# Autodesk Inventor assembly: Assembly_miscelatore
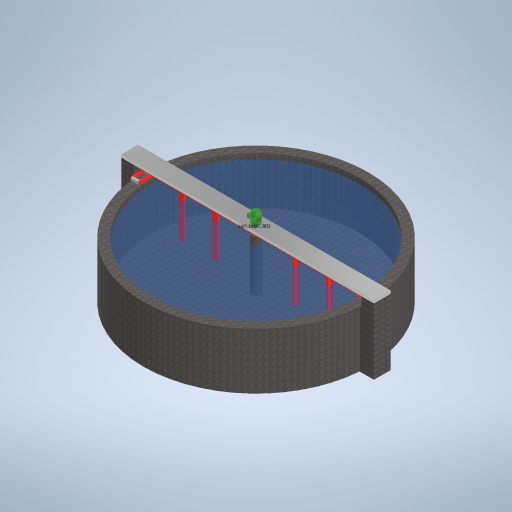
[picture p0: Inventor's stored thumbnail of the model, 512x512]
Saved by Autodesk Inventor 2024.2 (Build 282272000, 272)
## iProperties
Created: 2024-03-18
Part Number: Assembly_miscelatore
Document SubType Name: Assembly
Designer: feder
Author: feder
## Documents named in this file (9)
- C:\Users\feder\Desktop\FEM\PROJECT\Inventor\Assembly_miscelatore.iam
- C:\Users\feder\Desktop\FEM\PROJECT\Inventor\Vasca.ipt
- C:\Users\feder\Desktop\FEM\PROJECT\Inventor\Trave_e_Pale_inventor_coppia.ipt
- C:\Users\feder\Desktop\FEM\PROJECT\Inventor\trave_e_pale\Wheel60mm.ipt
- C:\Users\feder\Desktop\FEM\PROJECT\Inventor\trave_e_pale\Wheel120mm.ipt
- C:\Users\feder\Desktop\FEM\PROJECT\Inventor\Traversa_chiusura.ipt
- C:\Users\feder\Desktop\FEM\PROJECT\Inventor\water.ipt
- C:\Users\feder\Desktop\FEM\PROJECT\Inventor\7.5 KW 3000 rpm 132\7.5 KW 3000 rpm 132.ipt
- C:\Users\feder\Desktop\FEM\PROJECT\Inventor\Motor_beam_connection.ipt
## Components (10 placed, 8 different names)
1. Vasca:1 — Rotational:1, Rotational:6, Insert:2
2. water:1 — Rotational:1
3. Wheel120mm:1 — Rotational:4
4. Wheel120mm:2 — Rotational:3
5. Wheel60mm:1 — Rotational:2
6. Wheel60mm:2 — Rotational:5
7. Trave_e_Pale_inventor_coppia:2 — Rotational:2, Rotational:3, Rotational:4, Rotational:5, Rotational:6, Mate:1, Insert:1
8. Motor_beam_connection:1 — Mate:1, Insert:1
9. Traversa_chiusura:1 — Insert:2
10. 7.5 KW 3000 rpm 132:1
## Relationships (9: RevoluteJoint 6, Insert 2, Mate 1)
- Rotational:1 [RevoluteJoint]: Vasca:1 ↔ water:1
- Rotational:2 [RevoluteJoint]: Wheel60mm:1 ↔ Trave_e_Pale_inventor_coppia:2
- Rotational:3 [RevoluteJoint]: Wheel120mm:2 ↔ Trave_e_Pale_inventor_coppia:2
- Rotational:4 [RevoluteJoint]: Wheel120mm:1 ↔ Trave_e_Pale_inventor_coppia:2
- Rotational:5 [RevoluteJoint]: Wheel60mm:2 ↔ Trave_e_Pale_inventor_coppia:2
- Rotational:6 [RevoluteJoint]: Vasca:1 ↔ Trave_e_Pale_inventor_coppia:2
- Mate:1: Trave_e_Pale_inventor_coppia:2 ↔ Motor_beam_connection:1
- Insert:1: Trave_e_Pale_inventor_coppia:2 ↔ Motor_beam_connection:1
- Insert:2: Vasca:1 ↔ Traversa_chiusura:1
